# Autodesk Inventor assembly: левый привод_MIR
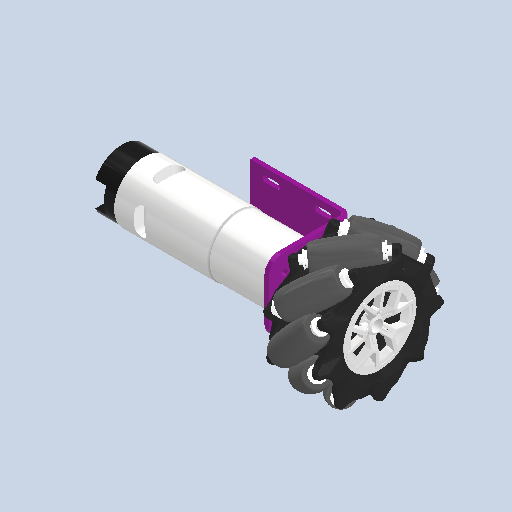
[picture p0: Inventor's stored thumbnail of the model, 512x512]
Saved by Autodesk Inventor 2025 (Build 290162000, 162)
## iProperties
Created: 2025-02-16
Part Number: левый привод_MIR
Document SubType Name: Assembly
Designer: volko
Author: volko
## Documents named in this file (5)
- C:\Users\volko\Desktop\диплом\Модели\детали\левый привод_MIR.iam
- C:\Users\volko\Desktop\диплом\Модели\детали\CHP-42GP-775 ABHL_MIR_MIR.ipt
- C:\Users\volko\Desktop\диплом\Модели\детали\кронштейн_MIR_MIR.ipt
- C:\Users\volko\Desktop\диплом\Модели\детали\переходная втулка_MIR_MIR.ipt
- C:\Users\volko\Desktop\диплом\Модели\Mecanum wheel - left\Mecanum wheel - left_MIR.iam
## Components (4 placed, 4 different names)
1. CHP-42GP-775 ABHL_MIR_MIR:1 — Заподлицо:1, Совмещение:2, Совмещение:1, Совмещение:7, Совмещение:6, Совмещение:5, Совмещение:4, Совмещение:3
2. кронштейн_MIR_MIR:1 — Совмещение:7, Совмещение:6, Совмещение:5
3. переходная втулка_MIR_MIR:1 — Совмещение:4, Совмещение:3, Совмещение:10, Совмещение:9, Совмещение:8
4. Mecanum wheel - left_MIR:1 [sub-assembly] — Совмещение:10, Совмещение:9, Совмещение:8
## Relationships (11: Mate 10, Flush 1)
- Заподлицо:1 [Flush]: CHP-42GP-775 ABHL_MIR_MIR:1
- Совмещение:2 [Mate]: CHP-42GP-775 ABHL_MIR_MIR:1
- Совмещение:1 [Mate]: CHP-42GP-775 ABHL_MIR_MIR:1
- Совмещение:7 [Mate]: CHP-42GP-775 ABHL_MIR_MIR:1 ↔ кронштейн_MIR_MIR:1
- Совмещение:6 [Mate]: CHP-42GP-775 ABHL_MIR_MIR:1 ↔ кронштейн_MIR_MIR:1
- Совмещение:5 [Mate]: CHP-42GP-775 ABHL_MIR_MIR:1 ↔ кронштейн_MIR_MIR:1
- Совмещение:4 [Mate]: CHP-42GP-775 ABHL_MIR_MIR:1 ↔ переходная втулка_MIR_MIR:1
- Совмещение:3 [Mate]: CHP-42GP-775 ABHL_MIR_MIR:1 ↔ переходная втулка_MIR_MIR:1
- Совмещение:10 [Mate]: переходная втулка_MIR_MIR:1 ↔ Mecanum wheel - left_MIR:1
- Совмещение:9 [Mate]: переходная втулка_MIR_MIR:1 ↔ Mecanum wheel - left_MIR:1
- Совмещение:8 [Mate]: переходная втулка_MIR_MIR:1 ↔ Mecanum wheel - left_MIR:1
